# Autodesk Inventor assembly: 1_Base
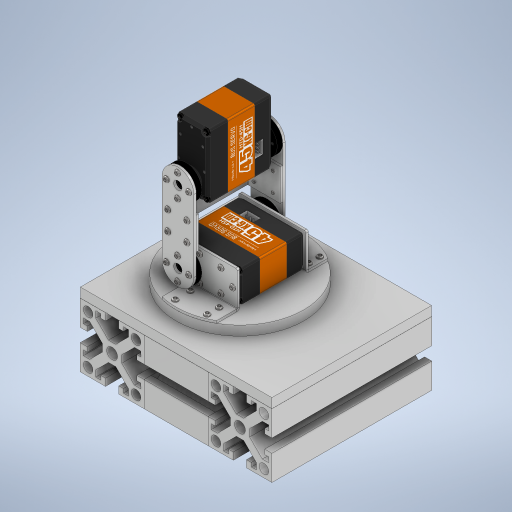
[picture p0: Inventor's stored thumbnail of the model, 512x512]
Saved by Autodesk Inventor 2024.1 (Build 281209000, 209)
## iProperties
Created: 2023-08-24
Part Number: 1_Base
Document SubType Name: Assembly
Designer: chanh
Author: chanh
## Documents named in this file (23)
- C:\Users\chanh\OneDrive - 연세대학교 (Yonsei University)\로봇\Humanoid\Roboin Humanoid Project\Inventor\rh_plus_7_axis_robot_arm_hardware\Assembly\2_Arm.iam
- C:\Users\chanh\OneDrive - 연세대학교 (Yonsei University)\로봇\Humanoid\Roboin Humanoid Project\Inventor\rh_plus_7_axis_robot_arm_hardware\Part\HTD-45H, Horn\HTD-45H\HTD-45H.ipt
- C:\Users\chanh\OneDrive - 연세대학교 (Yonsei University)\로봇\Humanoid\Roboin Humanoid Project\Inventor\rh_plus_7_axis_robot_arm_hardware\Part\Frame\axis_1_top_frame.ipt
- C:\Users\chanh\OneDrive - 연세대학교 (Yonsei University)\로봇\Humanoid\Roboin Humanoid Project\Inventor\rh_plus_7_axis_robot_arm_hardware\Part\Other Parts\Aluminum_Profile_4040_100.14mm_top.ipt
- C:\Users\chanh\OneDrive - 연세대학교 (Yonsei University)\로봇\Humanoid\Roboin Humanoid Project\Inventor\rh_plus_7_axis_robot_arm_hardware\Part\Other Parts\Aluminum_Profile_4040_40.10mm_right.ipt
- C:\Users\chanh\OneDrive - 연세대학교 (Yonsei University)\로봇\Humanoid\Roboin Humanoid Project\Inventor\rh_plus_7_axis_robot_arm_hardware\Part\Other Parts\Aluminum_Profile_4040_40.10mm_left.ipt
- C:\Users\chanh\OneDrive - 연세대학교 (Yonsei University)\로봇\Humanoid\Roboin Humanoid Project\Inventor\rh_plus_7_axis_robot_arm_hardware\Part\Other Parts\Aluminum_Profile_4040_100.14mm_bottom.ipt
- C:\Users\chanh\OneDrive - 연세대학교 (Yonsei University)\로봇\Humanoid\Roboin Humanoid Project\Inventor\rh_plus_7_axis_robot_arm_hardware\Part\HTD-45H, Horn\HTD-45H\M2x32.ipt
- C:\Users\chanh\OneDrive - 연세대학교 (Yonsei University)\로봇\Humanoid\Roboin Humanoid Project\Inventor\rh_plus_7_axis_robot_arm_hardware\Part\HTD-45H, Horn\Horn\Top Horn.ipt
- C:\Users\chanh\OneDrive - 연세대학교 (Yonsei University)\로봇\Humanoid\Roboin Humanoid Project\Inventor\rh_plus_7_axis_robot_arm_hardware\Part\Bolt, Bearing\M2x6 Round Bolt.ipt
- C:\Users\chanh\OneDrive - 연세대학교 (Yonsei University)\로봇\Humanoid\Roboin Humanoid Project\Inventor\rh_plus_7_axis_robot_arm_hardware\Part\Bolt, Bearing\M2x35 Round Bolt.ipt
- C:\Users\chanh\OneDrive - 연세대학교 (Yonsei University)\로봇\Humanoid\Roboin Humanoid Project\Inventor\rh_plus_7_axis_robot_arm_hardware\Part\Frame\axis_2_bottom_frame.ipt
- C:\Users\chanh\OneDrive - 연세대학교 (Yonsei University)\로봇\Humanoid\Roboin Humanoid Project\Inventor\rh_plus_7_axis_robot_arm_hardware\Part\Bolt, Bearing\AXK5070+AS Bearing.ipt
- C:\Users\chanh\OneDrive - 연세대학교 (Yonsei University)\로봇\Humanoid\Roboin Humanoid Project\Inventor\rh_plus_7_axis_robot_arm_hardware\Part\Bolt, Bearing\M2x6 Bolt.ipt
- C:\Users\chanh\OneDrive - 연세대학교 (Yonsei University)\로봇\Humanoid\Roboin Humanoid Project\Inventor\rh_plus_7_axis_robot_arm_hardware\Part\HTD-45H, Horn\HTD-45H\HTD-45H.iam
- C:\Users\chanh\OneDrive - 연세대학교 (Yonsei University)\로봇\Humanoid\Roboin Humanoid Project\Inventor\rh_plus_7_axis_robot_arm_hardware\Part\HTD-45H, Horn\Horn\M3x6.ipt
- C:\Users\chanh\OneDrive - 연세대학교 (Yonsei University)\로봇\Humanoid\Roboin Humanoid Project\Inventor\rh_plus_7_axis_robot_arm_hardware\Part\Frame\axis_2_bottom_L_frame(top).ipt
- C:\Users\chanh\OneDrive - 연세대학교 (Yonsei University)\로봇\Humanoid\Roboin Humanoid Project\Inventor\rh_plus_7_axis_robot_arm_hardware\Part\Frame\axis_2_bottom_L_frame(bottom).ipt
- C:\Users\chanh\OneDrive - 연세대학교 (Yonsei University)\로봇\Humanoid\Roboin Humanoid Project\Inventor\rh_plus_7_axis_robot_arm_hardware\Part\HTD-45H, Horn\Horn\Bottom Horn.ipt
- C:\Users\chanh\OneDrive - 연세대학교 (Yonsei University)\로봇\Humanoid\Roboin Humanoid Project\Inventor\rh_plus_7_axis_robot_arm_hardware\Part\Bolt, Bearing\M2x4 Round Bolt.ipt
- C:\Users\chanh\OneDrive - 연세대학교 (Yonsei University)\로봇\Humanoid\Roboin Humanoid Project\Inventor\rh_plus_7_axis_robot_arm_hardware\Part\Frame\axis_3_bottom_frame(top).ipt
- C:\Users\chanh\OneDrive - 연세대학교 (Yonsei University)\로봇\Humanoid\Roboin Humanoid Project\Inventor\rh_plus_7_axis_robot_arm_hardware\Part\Frame\axis_3_bottom_frame(bottom).ipt
- C:\Users\chanh\OneDrive - 연세대학교 (Yonsei University)\로봇\Humanoid\Roboin Humanoid Project\Inventor\rh_plus_7_axis_robot_arm_hardware\Part\Frame\axis_3_bottom_frame(middle).ipt
## Components (79 placed, 21 different names)
1. M2x4 Round Bolt:22 — Rigid:50
2. M2x4 Round Bolt:23 — Rigid:51
3. M2x4 Round Bolt:24 — Rigid:52
4. M2x4 Round Bolt:25 — Rigid:49
5. M2x4 Round Bolt:26 — Rigid:53
6. M2x4 Round Bolt:27 — Rigid:54
7. M2x4 Round Bolt:28 — Rigid:55
8. M2x4 Round Bolt:29 — Rigid:56
9. M2x4 Round Bolt:30 — Rigid:57
10. M2x4 Round Bolt:31 — Rigid:58
11. M2x4 Round Bolt:32 — Rigid:59
12. M2x4 Round Bolt:33 — Rigid:60
13. M2x4 Round Bolt:34 — Rigid:61
14. M2x4 Round Bolt:35 — Rigid:62
15. M2x4 Round Bolt:36 — Rigid:63
16. M2x4 Round Bolt:37 — Rigid:64
17. M2x4 Round Bolt:38 — Rigid:65
18. M2x4 Round Bolt:39 — Rigid:66
19. M2x4 Round Bolt:40 — Rigid:67
20. M2x4 Round Bolt:41 — Rigid:68
21. M2x4 Round Bolt:42 — Rigid:69
22. M2x4 Round Bolt:43 — Rigid:70
23. M2x4 Round Bolt:44 — Rigid:71
24. M2x4 Round Bolt:45 — Rigid:72
25. Aluminum_Profile_4040_100.14mm_top:1 — Flush:13, Flush:14, Mate:2, Mate:3, Flush:15, Flush:16, Mate:4, Flush:17, Flush:18, Mate:6
26. Aluminum_Profile_4040_40.10mm_right:1 — Mate:3, Flush:15, Flush:16
27. Aluminum_Profile_4040_40.10mm_left:1 — Mate:4, Flush:17, Flush:18, Mate:5, Flush:20
28. Aluminum_Profile_4040_100.14mm_bottom:1 — Flush:19, Mate:5, Flush:20
29. HTD-45H:1 — Mate:1, Flush:1, Flush:2, Flush:12, Flush:13, Flush:14, Mate:2, Flush:19, Rigid:1, Rigid:2, Rotational:1, Mate:7, Mate:8
30. axis_1_top_frame:1 — Flush:11, Flush:12, Mate:6, Rigid:11, Rigid:12, Rigid:13, Rigid:14, Rigid:15, Rigid:16, Rigid:17, Mate:9
31. HTD-45H:2 [sub-assembly] — Flush:21, Mate:11, Flush:23, Flush:24, Mate:13, Mate:17, Rotational:2, Rotational:3
32. axis_2_bottom_frame:1 — Rigid:10, Rigid:18, Rigid:19, Rigid:20, Rigid:21, Flush:21, Mate:11, Mate:14
33. axis_2_bottom_L_frame(top):1 — Flush:23, Flush:24, Mate:13, Mate:14, Rigid:23, Rigid:24, Rigid:25, Rigid:26, Rigid:27, Rigid:28, Rigid:29, Rigid:30, Rigid:31
34. axis_2_bottom_L_frame(bottom):1 — Mate:17, Rigid:32, Rigid:33, Rigid:34, Rigid:35, Rigid:36, Rigid:37, Rigid:38, Rigid:39, Rigid:40, Rigid:41, Rigid:42, Rigid:43
35. HTD-45H:3 [sub-assembly] — Rotational:4, Rotational:5
36. axis_3_bottom_frame(top):1 — Rigid:44, Rigid:45, Rigid:48, Rigid:49, Rigid:50, Rigid:51, Rigid:52, Rigid:53, Rigid:54, Rigid:55, Rigid:56, Rigid:57, Rigid:58, Rigid:59, Rigid:60
37. axis_3_bottom_frame(middle):1 — Rigid:48
38. axis_3_bottom_frame(bottom):1 — Rigid:46, Rigid:47, Rigid:61, Rigid:62, Rigid:63, Rigid:64, Rigid:65, Rigid:66, Rigid:67, Rigid:68, Rigid:69, Rigid:70, Rigid:71, Rigid:72
39. M2x32:1 — Rigid:2
40. M2x32:2 — Rigid:1
41. Top Horn:1 — Rotational:1, Rigid:10, Rigid:22
42. M3x6:1 — Rigid:22
43. M2x6 Round Bolt:3 — Rigid:16
44. M2x6 Round Bolt:4 — Rigid:17
45. M2x6 Round Bolt:5 — Rigid:15
46. AXK5070+AS Bearing:1 — Mate:7, Mate:8, Mate:9
47. M2x6 Round Bolt:1 — Rigid:14
48. M2x6 Round Bolt:2 — Rigid:13
49. M2x35 Round Bolt:1 — Rigid:11
50. M2x35 Round Bolt:2 — Rigid:12
51. Bottom Horn:1 — Rotational:3, Rigid:47
52. Top Horn:2 — Rotational:2, Rigid:44
53. M2x6 Bolt:1 — Rigid:18
54. M2x6 Bolt:2 — Rigid:19
55. M2x6 Bolt:3 — Rigid:20
56. M2x6 Bolt:4 — Rigid:21
57. M2x4 Round Bolt:1 — Rigid:23
58. M2x4 Round Bolt:2 — Rigid:24
59. M2x4 Round Bolt:3 — Rigid:25
60. M2x4 Round Bolt:4 — Rigid:26
61. M2x4 Round Bolt:5 — Rigid:27
62. M2x4 Round Bolt:6 — Rigid:28
63. M2x4 Round Bolt:7 — Rigid:29
64. M2x4 Round Bolt:8 — Rigid:30
65. M2x4 Round Bolt:9 — Rigid:31
66. M2x4 Round Bolt:10 — Rigid:32
67. M2x4 Round Bolt:11 — Rigid:33
68. M2x4 Round Bolt:12 — Rigid:34
69. M2x4 Round Bolt:13 — Rigid:35
70. M2x4 Round Bolt:14 — Rigid:36
71. M2x4 Round Bolt:15 — Rigid:37
72. M2x4 Round Bolt:16 — Rigid:38
73. M2x4 Round Bolt:17 — Rigid:39
74. M2x4 Round Bolt:18 — Rigid:40
75. M2x4 Round Bolt:19 — Rigid:41
76. M2x4 Round Bolt:20 — Rigid:42
77. M2x4 Round Bolt:21 — Rigid:43
78. Bottom Horn:2 — Rotational:5, Rigid:46
79. Top Horn:3 — Rotational:4, Rigid:45
## Relationships (98: WeldJoint 65, Flush 15, Mate 13, RevoluteJoint 5)
- Mate:1: HTD-45H:1
- Flush:1: HTD-45H:1
- Flush:2: HTD-45H:1
- Flush:11: axis_1_top_frame:1
- Flush:12: HTD-45H:1 ↔ axis_1_top_frame:1
- Flush:13: Aluminum_Profile_4040_100.14mm_top:1 ↔ HTD-45H:1
- Flush:14: Aluminum_Profile_4040_100.14mm_top:1 ↔ HTD-45H:1
- Mate:2: Aluminum_Profile_4040_100.14mm_top:1 ↔ HTD-45H:1
- Mate:3: Aluminum_Profile_4040_100.14mm_top:1 ↔ Aluminum_Profile_4040_40.10mm_right:1
- Flush:15: Aluminum_Profile_4040_100.14mm_top:1 ↔ Aluminum_Profile_4040_40.10mm_right:1
- Flush:16: Aluminum_Profile_4040_100.14mm_top:1 ↔ Aluminum_Profile_4040_40.10mm_right:1
- Mate:4: Aluminum_Profile_4040_100.14mm_top:1 ↔ Aluminum_Profile_4040_40.10mm_left:1
- Flush:17: Aluminum_Profile_4040_100.14mm_top:1 ↔ Aluminum_Profile_4040_40.10mm_left:1
- Flush:18: Aluminum_Profile_4040_100.14mm_top:1 ↔ Aluminum_Profile_4040_40.10mm_left:1
- Flush:19: Aluminum_Profile_4040_100.14mm_bottom:1 ↔ HTD-45H:1
- Mate:5: Aluminum_Profile_4040_40.10mm_left:1 ↔ Aluminum_Profile_4040_100.14mm_bottom:1
- Flush:20: Aluminum_Profile_4040_40.10mm_left:1 ↔ Aluminum_Profile_4040_100.14mm_bottom:1
- Mate:6: Aluminum_Profile_4040_100.14mm_top:1 ↔ axis_1_top_frame:1
- Rigid:1 [WeldJoint]: HTD-45H:1 ↔ M2x32:2
- Rigid:2 [WeldJoint]: HTD-45H:1 ↔ M2x32:1
- Rotational:1 [RevoluteJoint]: HTD-45H:1 ↔ Top Horn:1
- Rigid:10 [WeldJoint]: axis_2_bottom_frame:1 ↔ Top Horn:1
- Rigid:11 [WeldJoint]: axis_1_top_frame:1 ↔ M2x35 Round Bolt:1
- Rigid:12 [WeldJoint]: axis_1_top_frame:1 ↔ M2x35 Round Bolt:2
- Rigid:13 [WeldJoint]: axis_1_top_frame:1 ↔ M2x6 Round Bolt:2
- Rigid:14 [WeldJoint]: axis_1_top_frame:1 ↔ M2x6 Round Bolt:1
- Rigid:15 [WeldJoint]: axis_1_top_frame:1 ↔ M2x6 Round Bolt:5
- Rigid:16 [WeldJoint]: axis_1_top_frame:1 ↔ M2x6 Round Bolt:3
- Rigid:17 [WeldJoint]: axis_1_top_frame:1 ↔ M2x6 Round Bolt:4
- Mate:7: HTD-45H:1 ↔ AXK5070+AS Bearing:1
- Mate:8: HTD-45H:1 ↔ AXK5070+AS Bearing:1
- Mate:9: axis_1_top_frame:1 ↔ AXK5070+AS Bearing:1
- Rigid:18 [WeldJoint]: axis_2_bottom_frame:1 ↔ M2x6 Bolt:1
- Rigid:19 [WeldJoint]: axis_2_bottom_frame:1 ↔ M2x6 Bolt:2
- Rigid:20 [WeldJoint]: axis_2_bottom_frame:1 ↔ M2x6 Bolt:3
- Rigid:21 [WeldJoint]: axis_2_bottom_frame:1 ↔ M2x6 Bolt:4
- Rigid:22 [WeldJoint]: Top Horn:1 ↔ M3x6:1
- Flush:21: HTD-45H:2 ↔ axis_2_bottom_frame:1
- Mate:11: HTD-45H:2 ↔ axis_2_bottom_frame:1
- Flush:23: HTD-45H:2 ↔ axis_2_bottom_L_frame(top):1
- Flush:24 (-1 mm): HTD-45H:2 ↔ axis_2_bottom_L_frame(top):1
- Mate:13: HTD-45H:2 ↔ axis_2_bottom_L_frame(top):1
- Mate:14: axis_2_bottom_frame:1 ↔ axis_2_bottom_L_frame(top):1
- Mate:17: HTD-45H:2 ↔ axis_2_bottom_L_frame(bottom):1
- Rotational:2 [RevoluteJoint]: HTD-45H:2 ↔ Top Horn:2
- Rotational:3 [RevoluteJoint]: HTD-45H:2 ↔ Bottom Horn:1
- Rigid:23 [WeldJoint]: axis_2_bottom_L_frame(top):1 ↔ M2x4 Round Bolt:1
- Rigid:24 [WeldJoint]: axis_2_bottom_L_frame(top):1 ↔ M2x4 Round Bolt:2
- Rigid:25 [WeldJoint]: axis_2_bottom_L_frame(top):1 ↔ M2x4 Round Bolt:3
- Rigid:26 [WeldJoint]: axis_2_bottom_L_frame(top):1 ↔ M2x4 Round Bolt:4
- Rigid:27 [WeldJoint]: axis_2_bottom_L_frame(top):1 ↔ M2x4 Round Bolt:5
- Rigid:28 [WeldJoint]: axis_2_bottom_L_frame(top):1 ↔ M2x4 Round Bolt:6
- Rigid:29 [WeldJoint]: axis_2_bottom_L_frame(top):1 ↔ M2x4 Round Bolt:7
- Rigid:30 [WeldJoint]: axis_2_bottom_L_frame(top):1 ↔ M2x4 Round Bolt:8
- Rigid:31 [WeldJoint]: axis_2_bottom_L_frame(top):1 ↔ M2x4 Round Bolt:9
- Rigid:32 [WeldJoint]: axis_2_bottom_L_frame(bottom):1 ↔ M2x4 Round Bolt:10
- Rigid:33 [WeldJoint]: axis_2_bottom_L_frame(bottom):1 ↔ M2x4 Round Bolt:11
- Rigid:34 [WeldJoint]: axis_2_bottom_L_frame(bottom):1 ↔ M2x4 Round Bolt:12
- Rigid:35 [WeldJoint]: axis_2_bottom_L_frame(bottom):1 ↔ M2x4 Round Bolt:13
- Rigid:36 [WeldJoint]: axis_2_bottom_L_frame(bottom):1 ↔ M2x4 Round Bolt:14
- Rigid:37 [WeldJoint]: axis_2_bottom_L_frame(bottom):1 ↔ M2x4 Round Bolt:15
- Rigid:38 [WeldJoint]: axis_2_bottom_L_frame(bottom):1 ↔ M2x4 Round Bolt:16
- Rigid:39 [WeldJoint]: axis_2_bottom_L_frame(bottom):1 ↔ M2x4 Round Bolt:17
- Rigid:40 [WeldJoint]: axis_2_bottom_L_frame(bottom):1 ↔ M2x4 Round Bolt:18
- Rigid:41 [WeldJoint]: axis_2_bottom_L_frame(bottom):1 ↔ M2x4 Round Bolt:19
- Rigid:42 [WeldJoint]: axis_2_bottom_L_frame(bottom):1 ↔ M2x4 Round Bolt:20
- Rigid:43 [WeldJoint]: axis_2_bottom_L_frame(bottom):1 ↔ M2x4 Round Bolt:21
- Rotational:4 [RevoluteJoint]: HTD-45H:3 ↔ Top Horn:3
- Rotational:5 [RevoluteJoint]: HTD-45H:3 ↔ Bottom Horn:2
- Rigid:44 [WeldJoint]: axis_3_bottom_frame(top):1 ↔ Top Horn:2
- Rigid:45 [WeldJoint]: axis_3_bottom_frame(top):1 ↔ Top Horn:3
- Rigid:46 [WeldJoint]: axis_3_bottom_frame(bottom):1 ↔ Bottom Horn:2
- Rigid:47 [WeldJoint]: axis_3_bottom_frame(bottom):1 ↔ Bottom Horn:1
- Rigid:48 [WeldJoint]: axis_3_bottom_frame(top):1 ↔ axis_3_bottom_frame(middle):1
- Rigid:49 [WeldJoint]: M2x4 Round Bolt:25 ↔ axis_3_bottom_frame(top):1
- Rigid:50 [WeldJoint]: M2x4 Round Bolt:22 ↔ axis_3_bottom_frame(top):1
- Rigid:51 [WeldJoint]: M2x4 Round Bolt:23 ↔ axis_3_bottom_frame(top):1
- Rigid:52 [WeldJoint]: M2x4 Round Bolt:24 ↔ axis_3_bottom_frame(top):1
- Rigid:53 [WeldJoint]: M2x4 Round Bolt:26 ↔ axis_3_bottom_frame(top):1
- Rigid:54 [WeldJoint]: M2x4 Round Bolt:27 ↔ axis_3_bottom_frame(top):1
- Rigid:55 [WeldJoint]: M2x4 Round Bolt:28 ↔ axis_3_bottom_frame(top):1
- Rigid:56 [WeldJoint]: M2x4 Round Bolt:29 ↔ axis_3_bottom_frame(top):1
- Rigid:57 [WeldJoint]: M2x4 Round Bolt:30 ↔ axis_3_bottom_frame(top):1
- Rigid:58 [WeldJoint]: M2x4 Round Bolt:31 ↔ axis_3_bottom_frame(top):1
- Rigid:59 [WeldJoint]: M2x4 Round Bolt:32 ↔ axis_3_bottom_frame(top):1
- Rigid:60 [WeldJoint]: M2x4 Round Bolt:33 ↔ axis_3_bottom_frame(top):1
- Rigid:61 [WeldJoint]: M2x4 Round Bolt:34 ↔ axis_3_bottom_frame(bottom):1
- Rigid:62 [WeldJoint]: M2x4 Round Bolt:35 ↔ axis_3_bottom_frame(bottom):1
- Rigid:63 [WeldJoint]: M2x4 Round Bolt:36 ↔ axis_3_bottom_frame(bottom):1
- Rigid:64 [WeldJoint]: M2x4 Round Bolt:37 ↔ axis_3_bottom_frame(bottom):1
- Rigid:65 [WeldJoint]: M2x4 Round Bolt:38 ↔ axis_3_bottom_frame(bottom):1
- Rigid:66 [WeldJoint]: M2x4 Round Bolt:39 ↔ axis_3_bottom_frame(bottom):1
- Rigid:67 [WeldJoint]: M2x4 Round Bolt:40 ↔ axis_3_bottom_frame(bottom):1
- Rigid:68 [WeldJoint]: M2x4 Round Bolt:41 ↔ axis_3_bottom_frame(bottom):1
- Rigid:69 [WeldJoint]: M2x4 Round Bolt:42 ↔ axis_3_bottom_frame(bottom):1
- Rigid:70 [WeldJoint]: M2x4 Round Bolt:43 ↔ axis_3_bottom_frame(bottom):1
- Rigid:71 [WeldJoint]: M2x4 Round Bolt:44 ↔ axis_3_bottom_frame(bottom):1
- Rigid:72 [WeldJoint]: M2x4 Round Bolt:45 ↔ axis_3_bottom_frame(bottom):1
